# Autodesk Inventor assembly: Intake Basic Piston - full
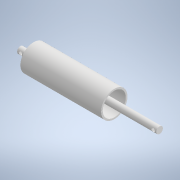
[picture p0: Inventor's stored thumbnail of the model, 180x180]
Saved by Autodesk Inventor 2020 (Build 240168000, 168)
## iProperties
Created: 2020-02-05
Part Number: Intake Basic Piston - full
Document SubType Name: Assembly
Designer: aidan
Author: aidan
## Documents named in this file (3)
- C:\Users\aidan\Desktop\T3 Robotics\CAD\Intake Basic Piston - full.iam
- C:\Users\aidan\Desktop\T3 Robotics\CAD\Intake Basic Piston - Outer.ipt
- C:\Users\aidan\Desktop\T3 Robotics\CAD\Intake Basic Piston - Inner.ipt
## Components (2 placed, 2 different names)
1. Intake Basic Piston - Outer:1 — Mate:1, Cylindrical:1
2. Intake Basic Piston - Inner:1 — Mate:1, Cylindrical:1
## Relationships (2: Mate 1, CylindricalJoint 1)
- Mate:1: Intake Basic Piston - Outer:1 ↔ Intake Basic Piston - Inner:1
- Cylindrical:1: Intake Basic Piston - Outer:1 ↔ Intake Basic Piston - Inner:1
